# Autodesk Inventor assembly: Gripper_assembly
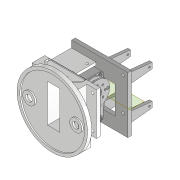
[picture p0: Inventor's stored thumbnail of the model, 180x180]
Saved by Autodesk Inventor 2022 (Build 260153000, 153)
## iProperties
Created: 2022-08-27
Part Number: Gripper_assembly
Document SubType Name: Assembly
Designer: dell
Author: dell
## Documents named in this file (6)
- D:\xxxx\Uni\Part IV\MECHENG_736\Gripper_project\Gripper_assembly.iam
- D:\xxxx\Uni\Part IV\MECHENG_736\Gripper_project\dovetail_female.ipt
- D:\xxxx\Uni\Part IV\MECHENG_736\Gripper_project\XM430.iam
- D:\xxxx\Uni\Part IV\MECHENG_736\Gripper_project\Mount_UR.ipt
- D:\xxxx\Uni\Part IV\MECHENG_736\Gripper_project\Motor_pulley.ipt
- D:\xxxx\Uni\Part IV\MECHENG_736\Gripper_project\Motor_plate.ipt
## Components (5 placed, 5 different names)
1. dovetail_female:1 — Mate:1, Mate:2, Flush:1, Mate:3, Mate:4
2. XM430:2 [sub-assembly] — Flush:1, Mate:3, Mate:4, Mate:5, Mate:6, Mate:7, Mate:8, Mate:9
3. Mount_UR:1 — Mate:1, Mate:2
4. Motor_pulley:1 — Mate:5, Mate:6
5. Motor_plate:1 — Mate:7, Mate:8, Mate:9
## Relationships (10: Mate 9, Flush 1)
- Mate:1: dovetail_female:1 ↔ Mount_UR:1
- Mate:2: dovetail_female:1 ↔ Mount_UR:1
- Flush:1: dovetail_female:1 ↔ XM430:2
- Mate:3: dovetail_female:1 ↔ XM430:2
- Mate:4: dovetail_female:1 ↔ XM430:2
- Mate:5: XM430:2 ↔ Motor_pulley:1
- Mate:6: XM430:2 ↔ Motor_pulley:1
- Mate:7: XM430:2 ↔ Motor_plate:1
- Mate:8: XM430:2 ↔ Motor_plate:1
- Mate:9: XM430:2 ↔ Motor_plate:1
